# Autodesk Inventor assembly: Cuvette-Sampleholder
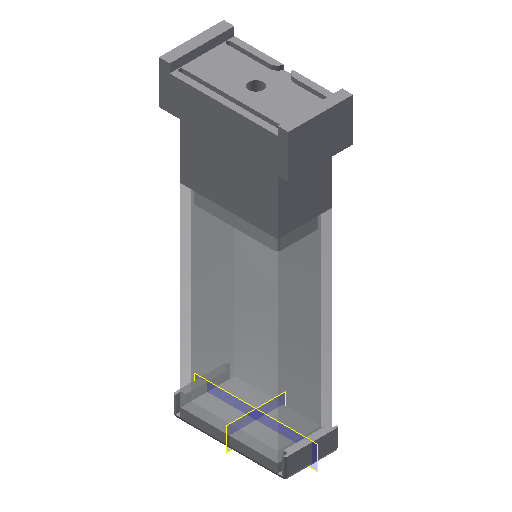
[picture p0: Inventor's stored thumbnail of the model, 512x512]
Saved by Autodesk Inventor 2023 (Build 270158000, 158)
## iProperties
Created: 2018-07-25
Part Number: Cuvette-Sampleholder
Document SubType Name: Assembly
Designer: voigt
Author: voigt
## Documents named in this file (4)
- C:\Users\Public\GitHub-public\benchtop-hardware\Benchtop\custom-parts\sample_handling\Deprecated\Cuvette-Sampleholder.iam
- C:\Users\Public\GitHub-public\benchtop-hardware\Benchtop\custom-parts\sample_handling\Deprecated\10x20mm_Cuvette_Top.ipt
- C:\Users\Public\GitHub-public\benchtop-hardware\Benchtop\CAD-model-Inventor\library\Portmann Instruments\UQ-205-10x20x45mm.ipt
- C:\Users\Public\GitHub-public\benchtop-hardware\Benchtop\custom-parts\sample_handling\Deprecated\10x20mm_Cuvette_Bottom.ipt
## Components (3 placed, 3 different names)
1. 10x20mm_Cuvette_Top:1 — Mate:1, Flush:1, Flush:2
2. UQ-205-10x20x45mm:1 — Mate:1, Flush:1, Flush:2, Flush:3
3. 10x20mm_Cuvette_Bottom:1 — Flush:3
## Relationships (4: Flush 3, Mate 1)
- Mate:1: 10x20mm_Cuvette_Top:1 ↔ UQ-205-10x20x45mm:1
- Flush:1: 10x20mm_Cuvette_Top:1 ↔ UQ-205-10x20x45mm:1
- Flush:2: 10x20mm_Cuvette_Top:1 ↔ UQ-205-10x20x45mm:1
- Flush:3: UQ-205-10x20x45mm:1 ↔ 10x20mm_Cuvette_Bottom:1
